# Autodesk Inventor assembly: Project_Box_Complete_Assembly
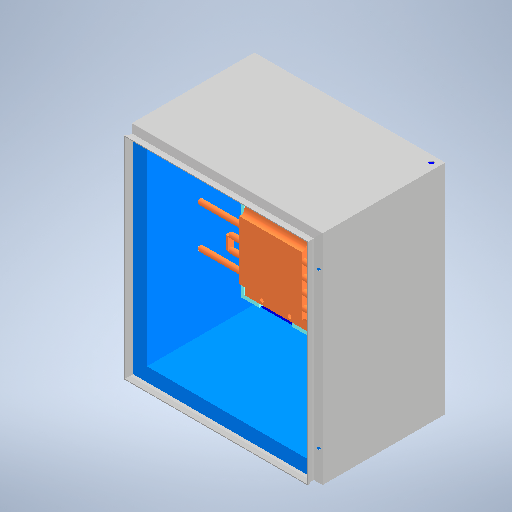
[picture p0: Inventor's stored thumbnail of the model, 512x512]
Saved by Autodesk Inventor 2025.2 (Build 292293000, 293)
## iProperties
Created: 2025-08-10
Part Number: Project_Box_Complete_Assembly
Document SubType Name: Assembly
Designer: cbast
Author: cbast
## Documents named in this file (7)
- C:\Users\cbast\OneDrive\Documents\GitHub\Smart-Pack-for-Advanced-Research-and-Control\variations\Camden\V0.2\Project_Box_Complete_Assembly.iam
- C:\Users\cbast\OneDrive\Documents\GitHub\Smart-Pack-for-Advanced-Research-and-Control\variations\Camden\V0.2\Project Box CAD\RITTAL Enclosure\F161410HC1.ipt
- C:\Users\cbast\OneDrive\Documents\GitHub\Smart-Pack-for-Advanced-Research-and-Control\variations\Camden\V0.2\Pillars_18650_Assembly.iam
- C:\Users\cbast\OneDrive\Documents\insulation.ipt
- C:\Users\cbast\OneDrive\Documents\insul2.ipt
- C:\Users\cbast\OneDrive\Documents\insul3.ipt
- C:\Users\cbast\OneDrive\Documents\Part8.ipt
## Components (8 placed, 6 different names)
1. F161410HC1:1 — Mate:1, Mate:2, Mate:3, Mate:4, Mate:5, Mate:7, Mate:8, Mate:10, Mate:11
2. Pillars_18650_Assembly:1 [sub-assembly] — Mate:16, Mate:17, Flush:1
3. insulation:1 — Mate:1, Mate:2, Mate:3, Mate:6, Mate:9, Mate:14, Mate:15, Mate:16
4. insul2:1 — Mate:4, Mate:5, Mate:6, Mate:12, Mate:17
5. insul2:2 — Mate:7, Mate:8, Mate:9, Mate:13
6. insul3:1 — Mate:11, Mate:12, Mate:14
7. insul3:2 — Mate:10, Mate:13, Mate:15
8. Part8:1 — Flush:1
## Relationships (18: Mate 17, Flush 1)
- Mate:1: F161410HC1:1 ↔ insulation:1
- Mate:2: F161410HC1:1 ↔ insulation:1
- Mate:3: F161410HC1:1 ↔ insulation:1
- Mate:4: F161410HC1:1 ↔ insul2:1
- Mate:5: F161410HC1:1 ↔ insul2:1
- Mate:6: insulation:1 ↔ insul2:1
- Mate:7: F161410HC1:1 ↔ insul2:2
- Mate:8: F161410HC1:1 ↔ insul2:2
- Mate:9: insulation:1 ↔ insul2:2
- Mate:10: F161410HC1:1 ↔ insul3:2
- Mate:11: F161410HC1:1 ↔ insul3:1
- Mate:12: insul2:1 ↔ insul3:1
- Mate:13: insul2:2 ↔ insul3:2
- Mate:14: insulation:1 ↔ insul3:1
- Mate:15: insulation:1 ↔ insul3:2
- Mate:16: Pillars_18650_Assembly:1 ↔ insulation:1
- Mate:17: Pillars_18650_Assembly:1 ↔ insul2:1
- Flush:1: Pillars_18650_Assembly:1 ↔ Part8:1
